# Autodesk Inventor assembly: fc16-005_GearMotorEncoder
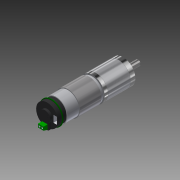
[picture p0: Inventor's stored thumbnail of the model, 180x180]
Saved by Autodesk Inventor 2016 SP1 (Build 200210100, 210)
## iProperties
Category: Electronics
Company: Autodesk Inc.
Created: 2015-11-26
Part Number: fc16-005_GearMotorEncoder
Document SubType Name: Assembly
Designer: Autodesk Inc.
Catalog Web Link: http://www.andymark.com/product-p/am-2971.htm
Vendor: AndyMark Inc.
Author: Autodesk Inc.
Keywords: FIRSTChoice
## Documents named in this file (3)
- D:\FIRST\FRC KOP 2016\FRC FIRSTChoice 2016\fc16-005_GearMotorEncoder.iam
- D:\FIRST\FRC KOP 2016\FRC FIRSTChoice 2016\fc16-004_GearMotor.ipt
- D:\FIRST\FRC KOP 2016\FRC FIRSTChoice 2016\Parts\Hall Effect Encoder for PG Gearboxes.ipt
## Components (2 placed, 2 different names)
1. fc16-004_GearMotor:1 — Insert:1, Angle:1
2. Hall Effect Encoder for PG Gearboxes:1 — Insert:1, Angle:1
## Relationships (2: Insert 1, Angle 1)
- Insert:1: fc16-004_GearMotor:1 ↔ Hall Effect Encoder for PG Gearboxes:1
- Angle:1 (0 deg): fc16-004_GearMotor:1 ↔ Hall Effect Encoder for PG Gearboxes:1
